# Autodesk Inventor assembly: ShooterAssembly_NERDS
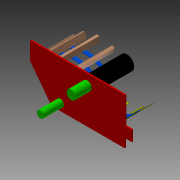
[picture p0: Inventor's stored thumbnail of the model, 180x180]
Saved by Autodesk Inventor 2014 (Build 180170000, 170)
## iProperties
Created: 2016-01-30
Part Number: ShooterAssembly_NERDS
Document SubType Name: Assembly
Designer: bermudezr
Author: bermudezr
## Documents named in this file (11)
- Z:\Nerds_1726\Robot\Shooting Mechanism\ShooterAssembly_NERDS.iam
- Z:\Nerds_1726\Robot\Shooting Mechanism\ShooterMountLeft_NERDS.ipt
- Z:\Nerds_1726\Robot\Shooting Mechanism\ShooterMountRight_NERDS.ipt
- Z:\Nerds_1726\Robot\Shooting Mechanism\Shooter_RollerTop.ipt
- Z:\Nerds_1726\Robot\Shooting Mechanism\Shooter_LowerMotor.ipt
- Z:\Nerds_1726\Robot\Shooting Mechanism\Shooter_LoadingRail.ipt
- Z:\Nerds_1726\Robot\Shooting Mechanism\Shooter_ShootingRail.ipt
- Z:\Nerds_1726\Robot\Chassis\SmallMotor_NERDS.ipt
- Z:\Nerds_1726\Robot\Chassis\Chassis_Motor.ipt
- Z:\Nerds_1726\Robot\Shooting Mechanism\RailMount1x2_NERDS.ipt
- Z:\Nerds_1726\Robot\Shooting Mechanism\RailMountMetal_NERDS.ipt
## Components (18 placed, 10 different names)
1. ShooterMountLeft_NERDS:1 — Flush:1, Flush:2, Mate:1, Mate:2, Mate:4, Mate:5
2. ShooterMountRight_NERDS:1 — Flush:1, Flush:2, Mate:1, Mate:3, Mate:12, Mate:14, Insert:1, Insert:2, Mate:17, Mate:18, Mate:19, Mate:20, Mate:21, Mate:22, Mate:23, Mate:24
3. Shooter_RollerTop:1 — Mate:2, Mate:5, Mate:9, Mate:10
4. Shooter_LowerMotor:1 — Mate:3, Mate:4, Mate:6, Mate:7, Mate:13
5. Shooter_LoadingRail:1 — Mate:6, Mate:8, Flush:3, Flush:5, Tangent:1, Tangent:2, Tangent:3
6. Shooter_LoadingRail:2 — Mate:7, Mate:8, Flush:5, Mate:12, Tangent:4
7. Shooter_ShootingRail:1 — Mate:9, Mate:11, Flush:4, Mate:14, Tangent:7
8. Shooter_ShootingRail:2 — Mate:10, Mate:11, Flush:3, Flush:4, Mate:13, Tangent:5, Tangent:6, Tangent:8
9. SmallMotor_NERDS:1 — Insert:1
10. Chassis_Motor:1 — Insert:2
11. RailMount1x2_NERDS:1 — Mate:17, Tangent:1
12. RailMount1x2_NERDS:2 — Mate:18, Tangent:2
13. RailMount1x2_NERDS:3 — Mate:19, Tangent:3
14. RailMount1x2_NERDS:4 — Mate:20, Tangent:4
15. RailMountMetal_NERDS:1 — Mate:21, Tangent:7
16. RailMountMetal_NERDS:2 — Mate:22, Tangent:6
17. RailMountMetal_NERDS:3 — Mate:23, Tangent:5
18. RailMountMetal_NERDS:4 — Mate:24, Tangent:8
## Relationships (37: Mate 22, Tangent 8, Flush 5, Insert 2)
- Flush:1: ShooterMountLeft_NERDS:1 ↔ ShooterMountRight_NERDS:1
- Flush:2: ShooterMountLeft_NERDS:1 ↔ ShooterMountRight_NERDS:1
- Mate:1 (275.8186 mm): ShooterMountLeft_NERDS:1 ↔ ShooterMountRight_NERDS:1
- Mate:2: ShooterMountLeft_NERDS:1 ↔ Shooter_RollerTop:1
- Mate:3: ShooterMountRight_NERDS:1 ↔ Shooter_LowerMotor:1
- Mate:4: ShooterMountLeft_NERDS:1 ↔ Shooter_LowerMotor:1
- Mate:5: ShooterMountLeft_NERDS:1 ↔ Shooter_RollerTop:1
- Mate:6: Shooter_LowerMotor:1 ↔ Shooter_LoadingRail:1
- Mate:7: Shooter_LowerMotor:1 ↔ Shooter_LoadingRail:2
- Mate:8 (50.8 mm): Shooter_LoadingRail:1 ↔ Shooter_LoadingRail:2
- Mate:9: Shooter_RollerTop:1 ↔ Shooter_ShootingRail:1
- Mate:10: Shooter_RollerTop:1 ↔ Shooter_ShootingRail:2
- Mate:11 (50.8 mm): Shooter_ShootingRail:1 ↔ Shooter_ShootingRail:2
- Flush:3: Shooter_LoadingRail:1 ↔ Shooter_ShootingRail:2
- Flush:4: Shooter_ShootingRail:1 ↔ Shooter_ShootingRail:2
- Flush:5: Shooter_LoadingRail:1 ↔ Shooter_LoadingRail:2
- Mate:12: ShooterMountRight_NERDS:1 ↔ Shooter_LoadingRail:2
- Mate:13 (38.1 mm): Shooter_LowerMotor:1 ↔ Shooter_ShootingRail:2
- Mate:14 (76.2 mm): ShooterMountRight_NERDS:1 ↔ Shooter_ShootingRail:1
- Insert:1: ShooterMountRight_NERDS:1 ↔ SmallMotor_NERDS:1
- Insert:2: ShooterMountRight_NERDS:1 ↔ Chassis_Motor:1
- Mate:17: ShooterMountRight_NERDS:1 ↔ RailMount1x2_NERDS:1
- Tangent:1: Shooter_LoadingRail:1 ↔ RailMount1x2_NERDS:1
- Mate:18: ShooterMountRight_NERDS:1 ↔ RailMount1x2_NERDS:2
- Mate:19: ShooterMountRight_NERDS:1 ↔ RailMount1x2_NERDS:3
- Mate:20: ShooterMountRight_NERDS:1 ↔ RailMount1x2_NERDS:4
- Tangent:2: Shooter_LoadingRail:1 ↔ RailMount1x2_NERDS:2
- Tangent:3: Shooter_LoadingRail:1 ↔ RailMount1x2_NERDS:3
- Tangent:4: Shooter_LoadingRail:2 ↔ RailMount1x2_NERDS:4
- Mate:21: ShooterMountRight_NERDS:1 ↔ RailMountMetal_NERDS:1
- Mate:22: ShooterMountRight_NERDS:1 ↔ RailMountMetal_NERDS:2
- Mate:23: ShooterMountRight_NERDS:1 ↔ RailMountMetal_NERDS:3
- Tangent:5: Shooter_ShootingRail:2 ↔ RailMountMetal_NERDS:3
- Tangent:6: Shooter_ShootingRail:2 ↔ RailMountMetal_NERDS:2
- Tangent:7: Shooter_ShootingRail:1 ↔ RailMountMetal_NERDS:1
- Mate:24: ShooterMountRight_NERDS:1 ↔ RailMountMetal_NERDS:4
- Tangent:8: Shooter_ShootingRail:2 ↔ RailMountMetal_NERDS:4
